# Autodesk Inventor assembly: Y_Axis_LM3021
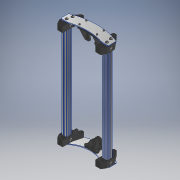
[picture p0: Inventor's stored thumbnail of the model, 180x180]
Saved by Autodesk Inventor 2020.2 (Build 242310000, 310)
## iProperties
Created: 2020-04-04
Part Number: Y_Axis_LM3021
Document SubType Name: Assembly
Designer: rah75
Author: rah75
## Documents named in this file (15)
- C:\Users\rah75\Documents\GitHub\LETU-Maker\CAD\Autodesk Inventor\Base_3001-5999\Y-Axis\Assemblies\Y_Axis_LM3021.iam
- C:\Users\rah75\Documents\GitHub\LETU-Maker\CAD\Autodesk Inventor\Base_3001-5999\Y-Axis\Printed_Parts\Y-Axis_Bearing_Mount_LM3012.ipt
- C:\Users\rah75\Documents\GitHub\LETU-Maker\CAD\Autodesk Inventor\Base_3001-5999\Y-Axis\Printed_Parts\Y-Axis_Foot_L_LM3014.ipt
- C:\Users\rah75\Documents\GitHub\LETU-Maker\CAD\Autodesk Inventor\Base_3001-5999\Y-Axis\Printed_Parts\Y-Axis_Motor_Mount_LM3017.ipt
- C:\Users\rah75\Documents\GitHub\LETU-Maker\CAD\Autodesk Inventor\Base_3001-5999\Y-Axis\Fabricated_Parts\Y-Axis_Motor_Plate_LM3018.ipt
- C:\Users\rah75\Documents\GitHub\LETU-Maker\CAD\Autodesk Inventor\Base_3001-5999\Y-Axis\Printed_Parts\Y-Axis_Foot_R_LM3016.ipt
- C:\Users\rah75\Documents\GitHub\LETU-Maker\CAD\Autodesk Inventor\Base_3001-5999\Y-Axis\Fabricated_Parts\Y-Axis_Extrusion_20x20x400mm_LM3020.ipt
- C:\Users\rah75\Documents\GitHub\LETU-Maker\CAD\Autodesk Inventor\Base_3001-5999\Y-Axis\Fabricated_Parts\Y-Axis_Bearing_Plate_LM3019.ipt
- C:\Users\rah75\Documents\GitHub\LETU-Maker\CAD\Autodesk Inventor\Base_3001-5999\Y-Axis\Printed_Parts\Y-Axis_Foot_w_Tap_R_LM3015.ipt
- C:\Users\rah75\Documents\GitHub\LETU-Maker\CAD\Autodesk Inventor\Stock_Components_1001-2999\Fasteners\Screws\BHHD_m5x10_LM1042.ipt
- C:\Users\rah75\Documents\GitHub\LETU-Maker\CAD\Autodesk Inventor\Stock_Components_1001-2999\Fasteners\Washers_Spacers\washer_m5_LM1002.ipt
- C:\Users\rah75\Documents\GitHub\LETU-Maker\CAD\Autodesk Inventor\Stock_Components_1001-2999\Fasteners\Nuts\heat_insert_m5_LM1018.ipt
- C:\Users\rah75\Documents\GitHub\LETU-Maker\CAD\Autodesk Inventor\Stock_Components_1001-2999\Fasteners\Nuts\heat_insert_m3_LM1017.ipt
- C:\Users\rah75\Documents\GitHub\LETU-Maker\CAD\Autodesk Inventor\Stock_Components_1001-2999\Fasteners\Nuts\hex_nut_m3_LM1019.ipt
- C:\Users\rah75\Documents\GitHub\LETU-Maker\CAD\Autodesk Inventor\Stock_Components_1001-2999\Fasteners\Screws\SHCS_m3x10_LM1015.ipt
## Components (66 placed, 14 different names)
1. Y-Axis_Motor_Mount_LM3017:1 — Insert:1, Mate:1, Insert:54, Insert:55, Insert:56, Insert:57
2. Y-Axis_Motor_Plate_LM3018:1 — Insert:1, Mate:1, Insert:2, Insert:3, Insert:4, Insert:5, Insert:29, Insert:30, Insert:31, Insert:32, Insert:58, Insert:59, Insert:60, Insert:61
3. Y-Axis_Foot_L_LM3014:1 — Insert:2, Flush:1, Insert:35, Insert:41, Insert:44, Insert:47
4. Y-Axis_Foot_R_LM3016:1 — Insert:3, Flush:1, Insert:28, Insert:40, Insert:45, Insert:46
5. Y-Axis_Extrusion_20x20x400mm_LM3020:1 — Insert:5, Insert:6
6. Y-Axis_Extrusion_20x20x400mm_LM3020:2 — Insert:4, Mate:2
7. Y-Axis_Bearing_Plate_LM3019:1 — Insert:6, Mate:2, Insert:7, Insert:8, Insert:9, Mate:3, Insert:36, Insert:37, Insert:38, Insert:39, Insert:62, Insert:63, Insert:64, Insert:65
8. Y-Axis_Bearing_Mount_LM3012:1 — Insert:9, Mate:3, Insert:50, Insert:51, Insert:52, Insert:53
9. Y-Axis_Foot_L_LM3014:2 — Insert:8, Flush:2, Insert:27, Insert:34, Insert:43, Insert:48
10. Y-Axis_Foot_w_Tap_R_LM3015:1 — Insert:7, Flush:2, Insert:26, Insert:33, Insert:42, Insert:49
11. BHHD_m5x10_LM1042:1 — Insert:10
12. BHHD_m5x10_LM1042:2 — Insert:11
13. BHHD_m5x10_LM1042:3 — Insert:12
14. BHHD_m5x10_LM1042:4 — Insert:14
15. BHHD_m5x10_LM1042:5 — Insert:15
16. BHHD_m5x10_LM1042:6 — Insert:17
17. BHHD_m5x10_LM1042:7 — Insert:16
18. BHHD_m5x10_LM1042:8 — Insert:13
19. BHHD_m5x10_LM1042:9 — Insert:23
20. BHHD_m5x10_LM1042:10 — Insert:22
21. BHHD_m5x10_LM1042:11 — Insert:21
22. BHHD_m5x10_LM1042:12 — Insert:18
23. BHHD_m5x10_LM1042:13 — Insert:19
24. BHHD_m5x10_LM1042:14 — Insert:20
25. BHHD_m5x10_LM1042:15 — Insert:24
26. BHHD_m5x10_LM1042:16 — Insert:25
27. washer_m5_LM1002:1 — Insert:10, Insert:26
28. washer_m5_LM1002:2 — Insert:11, Insert:36
29. washer_m5_LM1002:3 — Insert:13, Insert:27
30. washer_m5_LM1002:4 — Insert:16, Insert:37
31. washer_m5_LM1002:5 — Insert:14, Insert:28
32. washer_m5_LM1002:6 — Insert:22, Insert:40
33. washer_m5_LM1002:7 — Insert:24, Insert:32
34. washer_m5_LM1002:8 — Insert:21, Insert:30
35. washer_m5_LM1002:9 — Insert:20, Insert:29
36. washer_m5_LM1002:10 — Insert:17, Insert:38
37. washer_m5_LM1002:11 — Insert:15, Insert:34
38. washer_m5_LM1002:12 — Insert:12, Insert:33
39. washer_m5_LM1002:13 — Insert:18, Insert:35
40. washer_m5_LM1002:14 — Insert:19, Insert:31
41. washer_m5_LM1002:15 — Insert:23, Insert:39
42. washer_m5_LM1002:16 — Insert:25, Insert:41
43. heat_insert_m5_LM1018:1 — Insert:44
44. heat_insert_m5_LM1018:2 — Insert:45
45. heat_insert_m5_LM1018:3 — Insert:43
46. heat_insert_m5_LM1018:4 — Insert:42
47. heat_insert_m3_LM1017:1 — Insert:49
48. heat_insert_m3_LM1017:2 — Insert:48
49. heat_insert_m3_LM1017:3 — Insert:47
50. heat_insert_m3_LM1017:4 — Insert:46
51. hex_nut_m3_LM1019:1 — Insert:56
52. hex_nut_m3_LM1019:2 — Insert:53
53. hex_nut_m3_LM1019:3 — Insert:52
54. hex_nut_m3_LM1019:4 — Insert:50
55. hex_nut_m3_LM1019:5 — Insert:51
56. hex_nut_m3_LM1019:6 — Insert:57
57. hex_nut_m3_LM1019:7 — Insert:55
58. hex_nut_m3_LM1019:8 — Insert:54
59. SHCS_m3x10_LM1015:1 — Insert:58
60. SHCS_m3x10_LM1015:2 — Insert:59
61. SHCS_m3x10_LM1015:3 — Insert:60
62. SHCS_m3x10_LM1015:4 — Insert:61
63. SHCS_m3x10_LM1015:5 — Insert:62
64. SHCS_m3x10_LM1015:6 — Insert:63
65. SHCS_m3x10_LM1015:7 — Insert:64
66. SHCS_m3x10_LM1015:8 — Insert:65
## Relationships (70: Insert 65, Mate 3, Flush 2)
- Insert:1: Y-Axis_Motor_Mount_LM3017:1 ↔ Y-Axis_Motor_Plate_LM3018:1
- Mate:1: Y-Axis_Motor_Mount_LM3017:1 ↔ Y-Axis_Motor_Plate_LM3018:1
- Insert:2: Y-Axis_Motor_Plate_LM3018:1 ↔ Y-Axis_Foot_L_LM3014:1
- Insert:3: Y-Axis_Motor_Plate_LM3018:1 ↔ Y-Axis_Foot_R_LM3016:1
- Flush:1: Y-Axis_Foot_L_LM3014:1 ↔ Y-Axis_Foot_R_LM3016:1
- Insert:4: Y-Axis_Motor_Plate_LM3018:1 ↔ Y-Axis_Extrusion_20x20x400mm_LM3020:2
- Insert:5: Y-Axis_Motor_Plate_LM3018:1 ↔ Y-Axis_Extrusion_20x20x400mm_LM3020:1
- Insert:6: Y-Axis_Extrusion_20x20x400mm_LM3020:1 ↔ Y-Axis_Bearing_Plate_LM3019:1
- Mate:2: Y-Axis_Extrusion_20x20x400mm_LM3020:2 ↔ Y-Axis_Bearing_Plate_LM3019:1
- Insert:7: Y-Axis_Bearing_Plate_LM3019:1 ↔ Y-Axis_Foot_w_Tap_R_LM3015:1
- Insert:8: Y-Axis_Bearing_Plate_LM3019:1 ↔ Y-Axis_Foot_L_LM3014:2
- Insert:9: Y-Axis_Bearing_Plate_LM3019:1 ↔ Y-Axis_Bearing_Mount_LM3012:1
- Flush:2: Y-Axis_Foot_L_LM3014:2 ↔ Y-Axis_Foot_w_Tap_R_LM3015:1
- Mate:3: Y-Axis_Bearing_Plate_LM3019:1 ↔ Y-Axis_Bearing_Mount_LM3012:1
- Insert:10: BHHD_m5x10_LM1042:1 ↔ washer_m5_LM1002:1
- Insert:11: BHHD_m5x10_LM1042:2 ↔ washer_m5_LM1002:2
- Insert:12: BHHD_m5x10_LM1042:3 ↔ washer_m5_LM1002:12
- Insert:13: BHHD_m5x10_LM1042:8 ↔ washer_m5_LM1002:3
- Insert:14: BHHD_m5x10_LM1042:4 ↔ washer_m5_LM1002:5
- Insert:15: BHHD_m5x10_LM1042:5 ↔ washer_m5_LM1002:11
- Insert:16: BHHD_m5x10_LM1042:7 ↔ washer_m5_LM1002:4
- Insert:17: BHHD_m5x10_LM1042:6 ↔ washer_m5_LM1002:10
- Insert:18: BHHD_m5x10_LM1042:12 ↔ washer_m5_LM1002:13
- Insert:19: BHHD_m5x10_LM1042:13 ↔ washer_m5_LM1002:14
- Insert:20: BHHD_m5x10_LM1042:14 ↔ washer_m5_LM1002:9
- Insert:21: BHHD_m5x10_LM1042:11 ↔ washer_m5_LM1002:8
- Insert:22: BHHD_m5x10_LM1042:10 ↔ washer_m5_LM1002:6
- Insert:23: BHHD_m5x10_LM1042:9 ↔ washer_m5_LM1002:15
- Insert:24: BHHD_m5x10_LM1042:15 ↔ washer_m5_LM1002:7
- Insert:25: BHHD_m5x10_LM1042:16 ↔ washer_m5_LM1002:16
- Insert:26: Y-Axis_Foot_w_Tap_R_LM3015:1 ↔ washer_m5_LM1002:1
- Insert:27: Y-Axis_Foot_L_LM3014:2 ↔ washer_m5_LM1002:3
- Insert:28: Y-Axis_Foot_R_LM3016:1 ↔ washer_m5_LM1002:5
- Insert:29: Y-Axis_Motor_Plate_LM3018:1 ↔ washer_m5_LM1002:9
- Insert:30: Y-Axis_Motor_Plate_LM3018:1 ↔ washer_m5_LM1002:8
- Insert:31: Y-Axis_Motor_Plate_LM3018:1 ↔ washer_m5_LM1002:14
- Insert:32: Y-Axis_Motor_Plate_LM3018:1 ↔ washer_m5_LM1002:7
- Insert:33: Y-Axis_Foot_w_Tap_R_LM3015:1 ↔ washer_m5_LM1002:12
- Insert:34: Y-Axis_Foot_L_LM3014:2 ↔ washer_m5_LM1002:11
- Insert:35: Y-Axis_Foot_L_LM3014:1 ↔ washer_m5_LM1002:13
- Insert:36: Y-Axis_Bearing_Plate_LM3019:1 ↔ washer_m5_LM1002:2
- Insert:37: Y-Axis_Bearing_Plate_LM3019:1 ↔ washer_m5_LM1002:4
- Insert:38: Y-Axis_Bearing_Plate_LM3019:1 ↔ washer_m5_LM1002:10
- Insert:39: Y-Axis_Bearing_Plate_LM3019:1 ↔ washer_m5_LM1002:15
- Insert:40: Y-Axis_Foot_R_LM3016:1 ↔ washer_m5_LM1002:6
- Insert:41: Y-Axis_Foot_L_LM3014:1 ↔ washer_m5_LM1002:16
- Insert:42: Y-Axis_Foot_w_Tap_R_LM3015:1 ↔ heat_insert_m5_LM1018:4
- Insert:43: Y-Axis_Foot_L_LM3014:2 ↔ heat_insert_m5_LM1018:3
- Insert:44: Y-Axis_Foot_L_LM3014:1 ↔ heat_insert_m5_LM1018:1
- Insert:45: Y-Axis_Foot_R_LM3016:1 ↔ heat_insert_m5_LM1018:2
- Insert:46: Y-Axis_Foot_R_LM3016:1 ↔ heat_insert_m3_LM1017:4
- Insert:47: Y-Axis_Foot_L_LM3014:1 ↔ heat_insert_m3_LM1017:3
- Insert:48: Y-Axis_Foot_L_LM3014:2 ↔ heat_insert_m3_LM1017:2
- Insert:49: Y-Axis_Foot_w_Tap_R_LM3015:1 ↔ heat_insert_m3_LM1017:1
- Insert:50: Y-Axis_Bearing_Mount_LM3012:1 ↔ hex_nut_m3_LM1019:4
- Insert:51: Y-Axis_Bearing_Mount_LM3012:1 ↔ hex_nut_m3_LM1019:5
- Insert:52: Y-Axis_Bearing_Mount_LM3012:1 ↔ hex_nut_m3_LM1019:3
- Insert:53: Y-Axis_Bearing_Mount_LM3012:1 ↔ hex_nut_m3_LM1019:2
- Insert:54: Y-Axis_Motor_Mount_LM3017:1 ↔ hex_nut_m3_LM1019:8
- Insert:55: Y-Axis_Motor_Mount_LM3017:1 ↔ hex_nut_m3_LM1019:7
- Insert:56: Y-Axis_Motor_Mount_LM3017:1 ↔ hex_nut_m3_LM1019:1
- Insert:57: Y-Axis_Motor_Mount_LM3017:1 ↔ hex_nut_m3_LM1019:6
- Insert:58: Y-Axis_Motor_Plate_LM3018:1 ↔ SHCS_m3x10_LM1015:1
- Insert:59: Y-Axis_Motor_Plate_LM3018:1 ↔ SHCS_m3x10_LM1015:2
- Insert:60: Y-Axis_Motor_Plate_LM3018:1 ↔ SHCS_m3x10_LM1015:3
- Insert:61: Y-Axis_Motor_Plate_LM3018:1 ↔ SHCS_m3x10_LM1015:4
- Insert:62: Y-Axis_Bearing_Plate_LM3019:1 ↔ SHCS_m3x10_LM1015:5
- Insert:63: Y-Axis_Bearing_Plate_LM3019:1 ↔ SHCS_m3x10_LM1015:6
- Insert:64: Y-Axis_Bearing_Plate_LM3019:1 ↔ SHCS_m3x10_LM1015:7
- Insert:65: Y-Axis_Bearing_Plate_LM3019:1 ↔ SHCS_m3x10_LM1015:8
